# Autodesk Inventor assembly: BBP
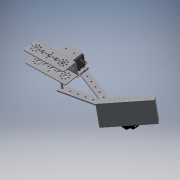
[picture p0: Inventor's stored thumbnail of the model, 180x180]
Saved by Autodesk Inventor 2016 (Build 200138000, 138)
## iProperties
Created: 2016-09-30
Part Number: BBP
Document SubType Name: Assembly
Designer: Delta
Author: Delta
## Documents named in this file (11)
- C:\Robotics\CAD\2016-17_CAD\BBP.iam
- C:\Robotics\CAD\COTSParts\Tetrix\Tetrix channel 160mm.ipt
- C:\Robotics\CAD\COTSParts\Tetrix\Tetrix bracket - single servo.ipt
- C:\Robotics\CAD\COTSParts\Actobotics\585 parts\585382.ipt
- C:\Robotics\CAD\COTSParts\Tetrix\Tetrix servo 180.ipt
- C:\Robotics\CAD\2015-16_CAD\Part5.ipt
- C:\Robotics\CAD\2015-16_CAD\Tetrix angle 144mm_3in.ipt
- C:\Robotics\CAD\COTSParts\ModernRobotics\45-2006_ODS.ipt
- C:\Robotics\CAD\COTSParts\Tetrix\Tetrix flat bar 7 in.ipt
- C:\Robotics\CAD\COTSParts\Tetrix\Tetrix flat bar 5.75.ipt
- C:\Robotics\CAD\2016-17_CAD\BBPBlock.ipt
## Components (11 placed, 10 different names)
1. Tetrix channel 160mm:2 — Insert:23, Insert:24, Insert:25
2. Tetrix bracket - single servo:1 — Insert:23, Insert:24, Flush:14, Flush:15, Mate:7
3. Tetrix servo 180:1 — Insert:21, Flush:14, Flush:15, Mate:7
4. 585382:5 — Insert:18, Mate:5, Flush:11, Flush:12, Mate:6
5. Part5:1 — Insert:25, Insert:26
6. Tetrix angle 144mm_3in:1 — Flush:7, Flush:8, Mate:3, Flush:9, Flush:10, Flush:11, Flush:12, Mate:6, Flush:16
7. Tetrix angle 144mm_3in:2 — Flush:7, Flush:8, Mate:3, Flush:9, Flush:10, Mate:8, Mate:9
8. 45-2006_ODS:1 — Insert:22
9. Tetrix flat bar 7 in:1 — Insert:18, Insert:22, Insert:26
10. Tetrix flat bar 5.75:1 — Insert:21, Mate:5
11. BBPBlock:1 — Mate:8, Flush:16, Mate:9
## Relationships (22: Flush 9, Insert 7, Mate 6)
- Flush:7: Tetrix angle 144mm_3in:1 ↔ Tetrix angle 144mm_3in:2
- Flush:8: Tetrix angle 144mm_3in:1 ↔ Tetrix angle 144mm_3in:2
- Mate:3: Tetrix angle 144mm_3in:1 ↔ Tetrix angle 144mm_3in:2
- Flush:9 (4.3434 mm): Tetrix angle 144mm_3in:1 ↔ Tetrix angle 144mm_3in:2
- Insert:18: 585382:5 ↔ Tetrix flat bar 7 in:1
- Insert:21: Tetrix servo 180:1 ↔ Tetrix flat bar 5.75:1
- Mate:5: 585382:5 ↔ Tetrix flat bar 5.75:1
- Flush:10: Tetrix angle 144mm_3in:1 ↔ Tetrix angle 144mm_3in:2
- Flush:11: 585382:5 ↔ Tetrix angle 144mm_3in:1
- Flush:12: 585382:5 ↔ Tetrix angle 144mm_3in:1
- Mate:6: 585382:5 ↔ Tetrix angle 144mm_3in:1
- Insert:22: 45-2006_ODS:1 ↔ Tetrix flat bar 7 in:1
- Insert:23: Tetrix channel 160mm:2 ↔ Tetrix bracket - single servo:1
- Insert:24: Tetrix channel 160mm:2 ↔ Tetrix bracket - single servo:1
- Flush:14: Tetrix bracket - single servo:1 ↔ Tetrix servo 180:1
- Flush:15: Tetrix bracket - single servo:1 ↔ Tetrix servo 180:1
- Mate:7: Tetrix bracket - single servo:1 ↔ Tetrix servo 180:1
- Insert:25: Tetrix channel 160mm:2 ↔ Part5:1
- Insert:26: Part5:1 ↔ Tetrix flat bar 7 in:1
- Mate:8: Tetrix angle 144mm_3in:2 ↔ BBPBlock:1
- Flush:16 (-12.7 mm): Tetrix angle 144mm_3in:1 ↔ BBPBlock:1
- Mate:9: Tetrix angle 144mm_3in:2 ↔ BBPBlock:1
